# Autodesk Inventor assembly: drivetrain-wheel
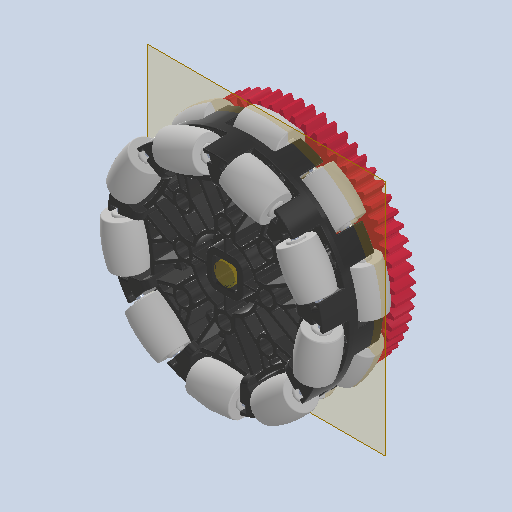
[picture p0: Inventor's stored thumbnail of the model, 512x512]
Saved by Autodesk Inventor 2025.2 (Build 292293000, 293)
## iProperties
Created: 2025-07-20
Part Number: drivetrain-wheel
Document SubType Name: Assembly
Designer: Exortions
Author: Exortions
## Documents named in this file (4)
- C:\3284b-cad-2025\Library\Custom Parts\drivetrain-wheel.iam
- C:\3284b-cad-2025\Library\VEX-CAD-Inventor-1.4.2\Motion\Wheels\Omni Wheel\2.75 Omni AS, No Insert.iam
- C:\3284b-cad-2025\Library\Custom Parts\halfcut-60t-gear.iam
- C:\3284b-cad-2025\Library\VEX-CAD-Inventor-1.4.2\Motion\Wheels\Omni Wheel.iam
## Components (2 placed, 2 different names)
1. 2.75 Omni AS, No Insert:1 [sub-assembly] — Insert:1, Mate:1
2. halfcut-60t-gear:1 [sub-assembly] — Insert:1, Mate:1
## Relationships (2: Insert 1, Mate 1)
- Insert:1 (6.35 mm): 2.75 Omni AS, No Insert:1 ↔ halfcut-60t-gear:1
- Mate:1: 2.75 Omni AS, No Insert:1 ↔ halfcut-60t-gear:1
